# Autodesk Inventor assembly: MotionBaseFixed
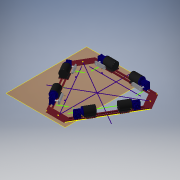
[picture p0: Inventor's stored thumbnail of the model, 180x180]
Saved by Autodesk Inventor 2016 (Build 200138000, 138)
## iProperties
Created: 2016-03-21
Part Number: MotionBaseFixed
Document SubType Name: Assembly
Designer: Mac
Author: Mac
## Documents named in this file (7)
- C:\Users\cutrones\Desktop\MotionBase\CAD\MotionBaseCAD\MotionBaseFixed2.iam
- C:\Users\cutrones\Desktop\MotionBase\CAD\MotionBaseCAD\Top.iam
- C:\Users\cutrones\Desktop\MotionBase\CAD\MotionBaseCAD\MotorRail.iam
- C:\Users\cutrones\Desktop\MotionBase\CAD\MotionBaseCAD\Triangle.ipt
- C:\Users\cutrones\Desktop\MotionBase\CAD\MotionBaseCAD\arm.ipt
- C:\Users\cutrones\Desktop\MotionBase\CAD\MotionBaseCAD\Bearing.ipt
- C:\Users\cutrones\Desktop\MotionBase\CAD\MotionBaseCAD\Triangle End.ipt
## Components (20 placed, 6 different names)
1. Top:1 [sub-assembly] — Mate:33, Mate:34, Mate:35, Mate:36, Mate:37, Mate:38, Angle:1
2. MotorRail:1 [sub-assembly] — Mate:3, Mate:6, Mate:18, Mate:29, Mate:30, Flush:10, Flush:11, Angle:1, Flush:14, Angle:2, Angle:3, Flush:26, Flush:30
3. MotorRail:2 [sub-assembly] — Mate:2, Mate:5, Mate:7, Mate:19, Mate:31, Mate:32, Flush:12, Flush:13, Flush:16, Flush:25, Flush:27
4. MotorRail:3 [sub-assembly] — Mate:1, Mate:4, Mate:20, Mate:27, Mate:28, Flush:8, Flush:9, Flush:17, Flush:19, Flush:28, Flush:29
5. Triangle:1 — Mate:1, Mate:2, Mate:3, Mate:4, Mate:5, Mate:6, Flush:1, Mate:8, Mate:9, Mate:10, Mate:11, Mate:12, Mate:13, Mate:14, Mate:15, Mate:16, Mate:17
6. arm:1 — Mate:21, Flush:2, Mate:28, Flush:8, Flush:20
7. Bearing:1 — Mate:21, Flush:2, Mate:34
8. arm:2 — Mate:29, Flush:11, Mate:42, Mate:43, Mate:44, Flush:22, Flush:23
9. Bearing:2 — Mate:36
10. arm:3 — Mate:31, Flush:12, Flush:23, Flush:24
11. Bearing:3 — Mate:37
12. arm:4 — Mate:30, Flush:10, Mate:45, Mate:46, Mate:47, Flush:21, Flush:22
13. Bearing:4 — Mate:35
14. arm:5 — Mate:32, Flush:13, Flush:24
15. Bearing:5 — Mate:38
16. arm:6 — Mate:27, Flush:9, Flush:20, Flush:21
17. Bearing:6 — Mate:33
18. Triangle End:1 — Flush:14, Flush:26, Flush:27
19. Triangle End:2 — Flush:16, Flush:17, Flush:25, Symmetry:1, Symmetry:2
20. Triangle End:3 — Flush:19, Flush:28, Flush:29, Flush:30, Symmetry:1, Symmetry:2
## Relationships (77: Mate 44, Flush 28, Angle 3, Symmetry 2)
- Mate:1: MotorRail:3 ↔ Triangle:1
- Mate:2: MotorRail:2 ↔ Triangle:1
- Mate:3: MotorRail:1 ↔ Triangle:1
- Mate:4: MotorRail:3 ↔ Triangle:1
- Mate:5: MotorRail:2 ↔ Triangle:1
- Mate:6: MotorRail:1 ↔ Triangle:1
- Flush:1: Triangle:1
- Mate:7: MotorRail:2
- Mate:8: Triangle:1
- Mate:9: Triangle:1
- Mate:10: Triangle:1
- Mate:11: Triangle:1
- Mate:12: Triangle:1
- Mate:13: Triangle:1
- Mate:14: Triangle:1
- Mate:15: Triangle:1
- Mate:16: Triangle:1
- Mate:17: Triangle:1
- Mate:18: MotorRail:1
- Mate:19: MotorRail:2
- Mate:20: MotorRail:3
- Mate:21: arm:1 ↔ Bearing:1
- Flush:2: arm:1 ↔ Bearing:1
- [Mate]: arm:2 ↔ Bearing:2
- [Flush]: arm:2 ↔ Bearing:2
- [Mate]: arm:3 ↔ Bearing:3
- [Flush]: arm:3 ↔ Bearing:3
- [Mate]: arm:4 ↔ Bearing:4
- [Flush]: arm:4 ↔ Bearing:4
- [Mate]: arm:5 ↔ Bearing:5
- [Flush]: arm:5 ↔ Bearing:5
- [Mate]: arm:6 ↔ Bearing:6
- [Flush]: arm:6 ↔ Bearing:6
- Mate:27: MotorRail:3 ↔ arm:6
- Mate:28: MotorRail:3 ↔ arm:1
- Mate:29: MotorRail:1 ↔ arm:2
- Mate:30: MotorRail:1 ↔ arm:4
- Mate:31: MotorRail:2 ↔ arm:3
- Mate:32: MotorRail:2 ↔ arm:5
- Flush:8: MotorRail:3 ↔ arm:1
- Flush:9: MotorRail:3 ↔ arm:6
- Flush:10: MotorRail:1 ↔ arm:4
- Flush:11: MotorRail:1 ↔ arm:2
- Flush:12: MotorRail:2 ↔ arm:3
- Flush:13: MotorRail:2 ↔ arm:5
- Mate:33: Top:1 ↔ Bearing:6
- Mate:34: Top:1 ↔ Bearing:1
- Mate:35: Top:1 ↔ Bearing:4
- Mate:36: Top:1 ↔ Bearing:2
- Mate:37: Top:1 ↔ Bearing:3
- Mate:38: Top:1 ↔ Bearing:5
- Angle:1 (0 deg): Top:1 ↔ MotorRail:1
- Flush:14: MotorRail:1 ↔ Triangle End:1
- Flush:16: MotorRail:2 ↔ Triangle End:2
- Flush:17: MotorRail:3 ↔ Triangle End:2
- Flush:19: MotorRail:3 ↔ Triangle End:3
- Mate:42: arm:2
- Mate:43: arm:2
- Mate:44: arm:2
- Angle:2 (0 deg): MotorRail:1
- Mate:45: arm:4
- Mate:46: arm:4
- Mate:47: arm:4
- Angle:3 (0 deg): MotorRail:1
- Flush:20: arm:1 ↔ arm:6
- Flush:21: arm:4 ↔ arm:6
- Flush:22: arm:2 ↔ arm:4
- Flush:23: arm:2 ↔ arm:3
- Flush:24: arm:3 ↔ arm:5
- Flush:25: MotorRail:2 ↔ Triangle End:2
- Flush:26: MotorRail:1 ↔ Triangle End:1
- Flush:27: MotorRail:2 ↔ Triangle End:1
- Flush:28: MotorRail:3 ↔ Triangle End:3
- Flush:29: MotorRail:3 ↔ Triangle End:3
- Flush:30: MotorRail:1 ↔ Triangle End:3
- Symmetry:1: Triangle End:2 ↔ Triangle End:3
- Symmetry:2: Triangle End:2 ↔ Triangle End:3
## Named parameters: d26_d24 = 0 mm, d27_d25 = 0 mm, d28_d24 = 0 mm, d29_d25 = 0 mm, d30_d24 = 0 mm, d31_d25 = 0 mm, d32_d24 = 0 mm, d33_d25 = 0 mm, d34_d24 = 0 mm, d35_d25 = 0 mm
